# Autodesk Inventor assembly: UpperBody_
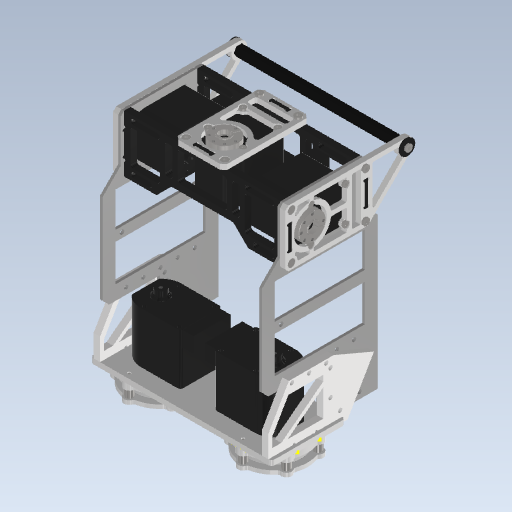
[picture p0: Inventor's stored thumbnail of the model, 512x512]
Saved by Autodesk Inventor 2020.4 (Build 244396000, 396)
## iProperties
Created: 2022-01-05
Part Number: UpperBody_
Document SubType Name: Assembly
Designer: Masato Kubotera
Author: Masato Kubotera
## Documents named in this file (20)
- C:\Users\Masato\Documents\Inventor\CIT Brains_Inventor\OpenPlatform_ver3_0 - ve4_1 branch\UpperBody\UpperBody_.iam
- C:\Users\Masato\Documents\Inventor\CIT Brains_Inventor\OpenPlatform_ver3_0 - ve4_1 branch\Ready_Made\KONDO\B3M-SC-1040-A.ipt
- C:\Users\Masato\Documents\Inventor\CIT Brains_Inventor\OpenPlatform_ver3_0 - ve4_1 branch\Ready_Made\KONDO\B3M-SC-1170-A.ipt
- C:\Users\Masato\Documents\Inventor\CIT Brains_Inventor\OpenPlatform_ver3_0 - ve4_1 branch\UpperBody\Trunk\Trunk_chest_frame.ipt
- C:\Users\Masato\Documents\Inventor\CIT Brains_Inventor\OpenPlatform_ver3_0 - ve4_1 branch\Ready_Made\InsertNut\IRU-304SW.ipt
- C:\Users\Masato\Documents\Inventor\CIT Brains_Inventor\OpenPlatform_ver3_0 - ve4_1 branch\UpperBody\Trunk\Trunk_neck_Upper_frame.ipt
- C:\Users\Masato\Documents\Inventor\CIT Brains_Inventor\OpenPlatform_ver3_0 - ve4_1 branch\Ready_Made\Screw\M2_6-15.ipt
- C:\Users\Masato\Documents\Inventor\CIT Brains_Inventor\OpenPlatform_ver3_0 - ve4_1 branch\Ready_Made\Screw\M3-6.ipt
- C:\Users\Masato\Documents\Inventor\CIT Brains_Inventor\OpenPlatform_ver3_0 - ve4_1 branch\Ready_Made\Screw\M3-8.ipt
- C:\Users\Masato\Documents\Inventor\CIT Brains_Inventor\OpenPlatform_ver3_0 - ve4_1 branch\UpperBody\Trunk\Trunk_shoulder_frame_.ipt
- C:\Users\Masato\Documents\Inventor\CIT Brains_Inventor\OpenPlatform_ver3_0 - ve4_1 branch\UpperBody\Trunk\Trunk_upper_side_frame.ipt
- C:\Users\Masato\Documents\Inventor\CIT Brains_Inventor\OpenPlatform_ver3_0 - ve4_1 branch\Ready_Made\Screw\M3-10.ipt
- C:\Users\Masato\Documents\Inventor\CIT Brains_Inventor\OpenPlatform_ver3_0 - ve4_1 branch\Ready_Made\ABLSBF7-133-M3-N3.ipt
- C:\Users\Masato\Documents\Inventor\CIT Brains_Inventor\OpenPlatform_ver3_0 - ve4_1 branch\UpperBody\Trunk\Trunk_shoulder_frame_MIR.ipt
- C:\Users\Masato\Documents\Inventor\CIT Brains_Inventor\OpenPlatform_ver3_0 - ve4_1 branch\Ready_Made\UUW-0312-10BH.ipt
- C:\Users\Masato\Documents\Inventor\CIT Brains_Inventor\OpenPlatform_ver3_0 - ve4_1 branch\UpperBody\Trunk\Trunk_lower_side_frame.ipt
- C:\Users\Masato\Documents\Inventor\CIT Brains_Inventor\OpenPlatform_ver3_0 - ve4_1 branch\UpperBody\Trunk\Trunk_waisit_frame_.ipt
- C:\Users\Masato\Documents\Inventor\CIT Brains_Inventor\OpenPlatform_ver3_0 - ve4_1 branch\UpperBody\Trunk\CrossRollerBearing\BearingUnit.iam
- C:\Users\Masato\Documents\Inventor\CIT Brains_Inventor\OpenPlatform_ver3_0 - ve4_1 branch\Ready_Made\KONDO\ClampHorn.ipt
- ClampHorn.ipt
## Components (65 placed, 18 different names)
1. B3M-SC-1040-A:1 — 挿入:13, 挿入:14, 挿入:15, 挿入:16, 挿入:95, 角度:2
2. B3M-SC-1040-A:2 — 挿入:41, 挿入:42, 挿入:43, 挿入:44, 挿入:96, 角度:3
3. B3M-SC-1040-A:3 — 挿入:61, 挿入:62, 挿入:63, 挿入:64, 挿入:97, 角度:4
4. B3M-SC-1170-A:1 — 挿入:87, 挿入:88
5. B3M-SC-1170-A:2 — 挿入:89, 挿入:90
6. Trunk_chest_frame:1 — 挿入:1, 挿入:2, 挿入:3, 挿入:4, 挿入:5, 挿入:6
7. Trunk_chest_frame:2 — 挿入:7, 挿入:8, 挿入:9, 挿入:10, 挿入:11, 挿入:12
8. IRU-304SW:1 — 挿入:1, 挿入:19
9. IRU-304SW:2 — 挿入:2, 挿入:20
10. IRU-304SW:3 — 挿入:3, 挿入:54
11. IRU-304SW:4 — 挿入:4, 挿入:55
12. IRU-304SW:5 — 挿入:5, 挿入:31
13. IRU-304SW:6 — 挿入:6, 挿入:32
14. IRU-304SW:7 — 挿入:7, 挿入:18
15. IRU-304SW:8 — 挿入:8, 挿入:17
16. IRU-304SW:9 — 挿入:9, 挿入:29
17. IRU-304SW:10 — 挿入:10, 挿入:30
18. IRU-304SW:11 — 挿入:11, 挿入:52
19. IRU-304SW:12 — 挿入:12, 挿入:53
20. Trunk_neck_Upper_frame:1 — 挿入:13, 挿入:14, 挿入:15, 挿入:16, 挿入:17, 挿入:18, 挿入:19, 挿入:20, 挿入:21, 挿入:22, 挿入:23, 挿入:24, 挿入:25, 挿入:26, 挿入:27, 挿入:28
21. M2_6-15:1 — 挿入:21
22. M2_6-15:2 — 挿入:22
23. M2_6-15:3 — 挿入:23
24. M2_6-15:4 — 挿入:24
25. M3-6:1 — 挿入:25
26. M3-6:2 — 挿入:26
27. M3-8:1 — 挿入:27
28. M3-8:2 — 挿入:28
29. Trunk_upper_side_frame:1 — 挿入:29, 挿入:30, 挿入:31, 挿入:32, 挿入:33, 挿入:34, 挿入:35, 挿入:36, 挿入:77, 挿入:78
30. Trunk_shoulder_frame_:1 — 挿入:33, 挿入:34, 挿入:35, 挿入:36, 挿入:37, 挿入:39, 挿入:38, 挿入:40, 挿入:41, 挿入:42, 挿入:43, 挿入:44, 挿入:47, 挿入:48, 挿入:49, 挿入:50, 角度:1, 挿入:51
31. M3-10:3 — 挿入:39
32. M3-10:4 — 挿入:40
33. M3-8:3 — 挿入:37
34. M3-8:4 — 挿入:38
35. M2_6-15:5 — 挿入:47
36. M2_6-15:6 — 挿入:48
37. M2_6-15:7 — 挿入:49
38. M2_6-15:8 — 挿入:50
39. ABLSBF7-133-M3-N3:1 — 角度:1, 挿入:51, 挿入:60, 挿入:73, 挿入:74
40. Trunk_upper_side_frame:2 — 挿入:52, 挿入:53, 挿入:54, 挿入:55, 挿入:56, 挿入:57, 挿入:58, 挿入:59, 挿入:79, 挿入:80
41. Trunk_shoulder_frame_MIR:1 — 挿入:56, 挿入:57, 挿入:58, 挿入:59, 挿入:60, 挿入:61, 挿入:62, 挿入:63, 挿入:64, 挿入:65, 挿入:66, 挿入:67, 挿入:68, 挿入:69, 挿入:70, 挿入:71, 挿入:72
42. M3-8:5 — 挿入:65
43. M3-8:6 — 挿入:66
44. M3-10:5 — 挿入:67
45. M3-10:6 — 挿入:68
46. M2_6-15:9 — 挿入:69
47. M2_6-15:10 — 挿入:70
48. M2_6-15:11 — 挿入:71
49. M2_6-15:12 — 挿入:72
50. UUW-0312-10BH:1 — 挿入:73, 挿入:75
51. UUW-0312-10BH:2 — 挿入:74, 挿入:76
52. M3-6:3 — 挿入:75
53. M3-6:4 — 挿入:76
54. Trunk_lower_side_frame:1 — 挿入:77, 挿入:78, 挿入:81, 挿入:82
55. Trunk_lower_side_frame:2 — 挿入:79, 挿入:80
56. Trunk_waisit_frame_:1 — 挿入:81, フラッシュ:2, 挿入:82, フラッシュ:3, フラッシュ:4, 挿入:83, 挿入:84, 挿入:85, 挿入:86, 挿入:87, 挿入:88, 挿入:89, 挿入:90, 挿入:91, 挿入:92, 挿入:93, 挿入:94
57. BearingUnit:1 [sub-assembly] — 挿入:83, 挿入:84
58. BearingUnit:2 [sub-assembly] — 挿入:85, 挿入:86
59. M2_6-15:13 — 挿入:91
60. M2_6-15:14 — 挿入:92
61. M2_6-15:15 — 挿入:93
62. M2_6-15:16 — 挿入:94
63. ClampHorn:1 — 挿入:95, 角度:2
64. ClampHorn:2 — 挿入:96, 角度:3
65. ClampHorn:3 — 挿入:97, 角度:4
## Relationships (102: Insert 95, Angle 4, Flush 3)
- 挿入:1 [Insert]: Trunk_chest_frame:1 ↔ IRU-304SW:1
- 挿入:2 [Insert]: Trunk_chest_frame:1 ↔ IRU-304SW:2
- 挿入:3 [Insert]: Trunk_chest_frame:1 ↔ IRU-304SW:3
- 挿入:4 [Insert]: Trunk_chest_frame:1 ↔ IRU-304SW:4
- 挿入:5 [Insert]: Trunk_chest_frame:1 ↔ IRU-304SW:5
- 挿入:6 [Insert]: Trunk_chest_frame:1 ↔ IRU-304SW:6
- 挿入:7 [Insert]: Trunk_chest_frame:2 ↔ IRU-304SW:7
- 挿入:8 [Insert]: Trunk_chest_frame:2 ↔ IRU-304SW:8
- 挿入:9 [Insert]: Trunk_chest_frame:2 ↔ IRU-304SW:9
- 挿入:10 [Insert]: Trunk_chest_frame:2 ↔ IRU-304SW:10
- 挿入:11 [Insert]: Trunk_chest_frame:2 ↔ IRU-304SW:11
- 挿入:12 [Insert]: Trunk_chest_frame:2 ↔ IRU-304SW:12
- 挿入:13 [Insert]: B3M-SC-1040-A:1 ↔ Trunk_neck_Upper_frame:1
- 挿入:14 [Insert]: B3M-SC-1040-A:1 ↔ Trunk_neck_Upper_frame:1
- 挿入:15 [Insert]: B3M-SC-1040-A:1 ↔ Trunk_neck_Upper_frame:1
- 挿入:16 [Insert]: B3M-SC-1040-A:1 ↔ Trunk_neck_Upper_frame:1
- 挿入:17 [Insert]: IRU-304SW:8 ↔ Trunk_neck_Upper_frame:1
- 挿入:18 [Insert]: IRU-304SW:7 ↔ Trunk_neck_Upper_frame:1
- 挿入:19 [Insert]: IRU-304SW:1 ↔ Trunk_neck_Upper_frame:1
- 挿入:20 [Insert]: IRU-304SW:2 ↔ Trunk_neck_Upper_frame:1
- 挿入:21 [Insert]: Trunk_neck_Upper_frame:1 ↔ M2_6-15:1
- 挿入:22 [Insert]: Trunk_neck_Upper_frame:1 ↔ M2_6-15:2
- 挿入:23 [Insert]: Trunk_neck_Upper_frame:1 ↔ M2_6-15:3
- 挿入:24 [Insert]: Trunk_neck_Upper_frame:1 ↔ M2_6-15:4
- 挿入:25 [Insert]: Trunk_neck_Upper_frame:1 ↔ M3-6:1
- 挿入:26 [Insert]: Trunk_neck_Upper_frame:1 ↔ M3-6:2
- 挿入:27 [Insert]: Trunk_neck_Upper_frame:1 ↔ M3-8:1
- 挿入:28 [Insert]: Trunk_neck_Upper_frame:1 ↔ M3-8:2
- 挿入:29 [Insert]: IRU-304SW:9 ↔ Trunk_upper_side_frame:1
- 挿入:30 [Insert]: IRU-304SW:10 ↔ Trunk_upper_side_frame:1
- 挿入:31 [Insert]: IRU-304SW:5 ↔ Trunk_upper_side_frame:1
- 挿入:32 [Insert]: IRU-304SW:6 ↔ Trunk_upper_side_frame:1
- 挿入:33 [Insert]: Trunk_upper_side_frame:1 ↔ Trunk_shoulder_frame_:1
- 挿入:34 [Insert]: Trunk_upper_side_frame:1 ↔ Trunk_shoulder_frame_:1
- 挿入:35 [Insert]: Trunk_upper_side_frame:1 ↔ Trunk_shoulder_frame_:1
- 挿入:36 [Insert]: Trunk_upper_side_frame:1 ↔ Trunk_shoulder_frame_:1
- 挿入:37 [Insert]: Trunk_shoulder_frame_:1 ↔ M3-8:3
- 挿入:39 [Insert]: Trunk_shoulder_frame_:1 ↔ M3-10:3
- 挿入:38 [Insert]: Trunk_shoulder_frame_:1 ↔ M3-8:4
- 挿入:40 [Insert]: Trunk_shoulder_frame_:1 ↔ M3-10:4
- 挿入:41 [Insert]: B3M-SC-1040-A:2 ↔ Trunk_shoulder_frame_:1
- 挿入:42 [Insert]: B3M-SC-1040-A:2 ↔ Trunk_shoulder_frame_:1
- 挿入:43 [Insert]: B3M-SC-1040-A:2 ↔ Trunk_shoulder_frame_:1
- 挿入:44 [Insert]: B3M-SC-1040-A:2 ↔ Trunk_shoulder_frame_:1
- 挿入:47 [Insert]: Trunk_shoulder_frame_:1 ↔ M2_6-15:5
- 挿入:48 [Insert]: Trunk_shoulder_frame_:1 ↔ M2_6-15:6
- 挿入:49 [Insert]: Trunk_shoulder_frame_:1 ↔ M2_6-15:7
- 挿入:50 [Insert]: Trunk_shoulder_frame_:1 ↔ M2_6-15:8
- 角度:1 [Angle] (0 deg): Trunk_shoulder_frame_:1 ↔ ABLSBF7-133-M3-N3:1
- 挿入:51 [Insert]: Trunk_shoulder_frame_:1 ↔ ABLSBF7-133-M3-N3:1
- 挿入:52 [Insert]: IRU-304SW:11 ↔ Trunk_upper_side_frame:2
- 挿入:53 [Insert]: IRU-304SW:12 ↔ Trunk_upper_side_frame:2
- 挿入:54 [Insert]: IRU-304SW:3 ↔ Trunk_upper_side_frame:2
- 挿入:55 [Insert]: IRU-304SW:4 ↔ Trunk_upper_side_frame:2
- 挿入:56 [Insert]: Trunk_upper_side_frame:2 ↔ Trunk_shoulder_frame_MIR:1
- 挿入:57 [Insert]: Trunk_upper_side_frame:2 ↔ Trunk_shoulder_frame_MIR:1
- 挿入:58 [Insert]: Trunk_upper_side_frame:2 ↔ Trunk_shoulder_frame_MIR:1
- 挿入:59 [Insert]: Trunk_upper_side_frame:2 ↔ Trunk_shoulder_frame_MIR:1
- 挿入:60 [Insert]: ABLSBF7-133-M3-N3:1 ↔ Trunk_shoulder_frame_MIR:1
- 挿入:61 [Insert]: B3M-SC-1040-A:3 ↔ Trunk_shoulder_frame_MIR:1
- 挿入:62 [Insert]: B3M-SC-1040-A:3 ↔ Trunk_shoulder_frame_MIR:1
- 挿入:63 [Insert]: B3M-SC-1040-A:3 ↔ Trunk_shoulder_frame_MIR:1
- 挿入:64 [Insert]: B3M-SC-1040-A:3 ↔ Trunk_shoulder_frame_MIR:1
- 挿入:65 [Insert]: Trunk_shoulder_frame_MIR:1 ↔ M3-8:5
- 挿入:66 [Insert]: Trunk_shoulder_frame_MIR:1 ↔ M3-8:6
- 挿入:67 [Insert]: Trunk_shoulder_frame_MIR:1 ↔ M3-10:5
- 挿入:68 [Insert]: Trunk_shoulder_frame_MIR:1 ↔ M3-10:6
- 挿入:69 [Insert]: Trunk_shoulder_frame_MIR:1 ↔ M2_6-15:9
- 挿入:70 [Insert]: Trunk_shoulder_frame_MIR:1 ↔ M2_6-15:10
- 挿入:71 [Insert]: Trunk_shoulder_frame_MIR:1 ↔ M2_6-15:11
- 挿入:72 [Insert]: Trunk_shoulder_frame_MIR:1 ↔ M2_6-15:12
- 挿入:73 [Insert]: ABLSBF7-133-M3-N3:1 ↔ UUW-0312-10BH:1
- 挿入:74 [Insert]: ABLSBF7-133-M3-N3:1 ↔ UUW-0312-10BH:2
- 挿入:75 [Insert]: UUW-0312-10BH:1 ↔ M3-6:3
- 挿入:76 [Insert]: UUW-0312-10BH:2 ↔ M3-6:4
- 挿入:77 [Insert]: Trunk_upper_side_frame:1 ↔ Trunk_lower_side_frame:1
- 挿入:78 [Insert]: Trunk_upper_side_frame:1 ↔ Trunk_lower_side_frame:1
- 挿入:79 [Insert]: Trunk_upper_side_frame:2 ↔ Trunk_lower_side_frame:2
- 挿入:80 [Insert]: Trunk_upper_side_frame:2 ↔ Trunk_lower_side_frame:2
- 挿入:81 [Insert]: Trunk_lower_side_frame:1 ↔ Trunk_waisit_frame_:1
- フラッシュ:2 [Flush]: Trunk_waisit_frame_:1
- 挿入:82 [Insert]: Trunk_lower_side_frame:1 ↔ Trunk_waisit_frame_:1
- フラッシュ:3 [Flush]: Trunk_waisit_frame_:1
- フラッシュ:4 [Flush]: Trunk_waisit_frame_:1
- 挿入:83 [Insert]: Trunk_waisit_frame_:1 ↔ BearingUnit:1
- 挿入:84 [Insert]: Trunk_waisit_frame_:1 ↔ BearingUnit:1
- 挿入:85 [Insert]: Trunk_waisit_frame_:1 ↔ BearingUnit:2
- 挿入:86 [Insert]: Trunk_waisit_frame_:1 ↔ BearingUnit:2
- 挿入:87 [Insert]: B3M-SC-1170-A:1 ↔ Trunk_waisit_frame_:1
- 挿入:88 [Insert]: B3M-SC-1170-A:1 ↔ Trunk_waisit_frame_:1
- 挿入:89 [Insert]: B3M-SC-1170-A:2 ↔ Trunk_waisit_frame_:1
- 挿入:90 [Insert]: B3M-SC-1170-A:2 ↔ Trunk_waisit_frame_:1
- 挿入:91 [Insert]: Trunk_waisit_frame_:1 ↔ M2_6-15:13
- 挿入:92 [Insert]: Trunk_waisit_frame_:1 ↔ M2_6-15:14
- 挿入:93 [Insert]: Trunk_waisit_frame_:1 ↔ M2_6-15:15
- 挿入:94 [Insert]: Trunk_waisit_frame_:1 ↔ M2_6-15:16
- 挿入:95 [Insert]: B3M-SC-1040-A:1 ↔ ClampHorn:1
- 挿入:96 [Insert]: B3M-SC-1040-A:2 ↔ ClampHorn:2
- 挿入:97 [Insert]: B3M-SC-1040-A:3 ↔ ClampHorn:3
- 角度:2 [Angle] (0 deg): B3M-SC-1040-A:1 ↔ ClampHorn:1
- 角度:3 [Angle] (0 deg): B3M-SC-1040-A:2 ↔ ClampHorn:2
- 角度:4 [Angle] (0 deg): B3M-SC-1040-A:3 ↔ ClampHorn:3
